# Autodesk Inventor assembly: HalfChassisAssem
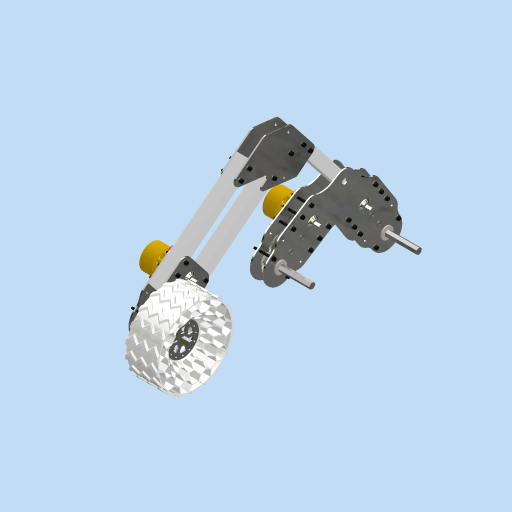
[picture p0: Inventor's stored thumbnail of the model, 512x512]
Saved by Autodesk Inventor 2023 (Build 270158000, 158)
## iProperties
Created: 2023-04-06
Part Number: HalfChassisAssem
Document SubType Name: Assembly
Designer: Dave
Mass: 5362.71 g
Surface Area: 20188.6 cm^2
Volume: 2426.63 cm^3
Density: 2.20995 g/cm^3
Author: Dave
## Documents named in this file (14)
- C:\Github\BehrendURC\CAD\Chassis V3\HalfChassisAssem.iam
- C:\Github\BehrendURC\CAD\Chassis V3\L3 Gearbox Assembly.iam
- C:\Github\BehrendURC\CAD\Chassis V3\L1 Gearbox Assembly.iam
- C:\Github\BehrendURC\CAD\Chassis V3\HipPivotPlate.ipt
- C:\Users\Dave\Documents\GitHub\BehrendURCMechanical\CAD\Chassis V3\aluminumextrusiontool.ipt
- C:\Github\BehrendURC\CAD\Chassis V3\aluminumextrusiontool\aluminumextrusiontool-17-10.6in.ipt
- C:\Github\BehrendURC\CAD\Chassis V3\aluminumextrusiontool\aluminumextrusiontool-17-13.31255in.ipt
- C:\Github\BehrendURC\CAD\Chassis V3\Pivot Files and Assembly\PivotAssembly.iam
- C:\Github\BehrendURC\CAD\Chassis V3\aluminumextrusiontool\aluminumextrusiontool-17-7.9.ipt
- C:\Github\BehrendURC\CAD\Chassis V3\91333A140_Low-Strength Steel Nylon-Insert Locknut.ipt
- C:\Github\BehrendURC\CAD\Chassis V3\90107A011_316 Stainless Steel Washer.ipt
- C:\Github\BehrendURC\CAD\Chassis V3\Bolt Nut Washer assem.iam
- C:\Github\BehrendURC\CAD\Chassis V3\Pivot Files and Assembly\91831A011_18-8 Stainless Steel Nylon-Insert Locknut (1).ipt
- C:\Github\BehrendURC\CAD\Chassis V3\Wheel\WheelAssembly_v9.iam
## Components (20 placed, 12 different names)
1. L3 Gearbox Assembly:1 [sub-assembly] — Mate:4, Tangent:2, Mate:10, Insert:1
2. L1 Gearbox Assembly:1 [sub-assembly] — Flush:2, Flush:3, Mate:1, Flush:6, Mate:2, Flush:7, Mate:3, Mate:11, Flush:13, Tangent:3, Mate:12, Mate:13, Flush:14
3. HipPivotPlate:1 — Flush:3, Flush:4, Flush:5, Mate:5, Insert:4
4. HipPivotPlate:2 — Flush:2, Flush:4, Flush:5, Mate:1, Flush:6, Mate:4, Flush:8, Tangent:1, Mate:6, Flush:9, Insert:6, Insert:7, Insert:9, Insert:10, Insert:11, Insert:12, Insert:14
5. aluminumextrusiontool-17-10.6in:1 — Mate:2, Flush:7, Mate:3
6. aluminumextrusiontool-17-7.9:2 — Mate:5, Flush:8, Tangent:1, Tangent:2, Mate:10
7. aluminumextrusiontool-17-13.31255in:3 — Mate:11, Flush:13, Tangent:3
8. PivotAssembly:2 [sub-assembly] — Insert:1, Insert:16
9. PivotAssembly:3 [sub-assembly] — Insert:6, Insert:15
10. 91333A140_Low-Strength Steel Nylon-Insert Locknut:1 — Insert:5
11. 90107A011_316 Stainless Steel Washer:1 — Insert:4, Insert:5
12. Bolt Nut Washer assem:1 [sub-assembly] — Insert:7
13. Bolt Nut Washer assem:3 [sub-assembly] — Insert:9
14. Bolt Nut Washer assem:4 [sub-assembly] — Insert:10
15. Bolt Nut Washer assem:5 [sub-assembly] — Insert:11
16. Bolt Nut Washer assem:6 [sub-assembly] — Insert:12
17. Bolt Nut Washer assem:8 [sub-assembly] — Insert:14
18. 91831A011_18-8 Stainless Steel Nylon-Insert Locknut (1):1 — Insert:15
19. 91831A011_18-8 Stainless Steel Nylon-Insert Locknut (1):2 — Insert:16
20. WheelAssembly_v9:1 [sub-assembly] — Mate:12, Mate:13, Flush:14
## Relationships (35: Insert 12, Flush 10, Mate 10, Tangent 3)
- Flush:2: L1 Gearbox Assembly:1 ↔ HipPivotPlate:2
- Flush:3: L1 Gearbox Assembly:1 ↔ HipPivotPlate:1
- Flush:4: HipPivotPlate:1 ↔ HipPivotPlate:2
- Flush:5: HipPivotPlate:1 ↔ HipPivotPlate:2
- Mate:1 (396 mm): L1 Gearbox Assembly:1 ↔ HipPivotPlate:2
- Flush:6: L1 Gearbox Assembly:1 ↔ HipPivotPlate:2
- Mate:2: L1 Gearbox Assembly:1 ↔ aluminumextrusiontool-17-10.6in:1
- Flush:7: L1 Gearbox Assembly:1 ↔ aluminumextrusiontool-17-10.6in:1
- Mate:3 (-76.2 mm): L1 Gearbox Assembly:1 ↔ aluminumextrusiontool-17-10.6in:1
- Mate:4 (216 mm): L3 Gearbox Assembly:1 ↔ HipPivotPlate:2
- Mate:5: HipPivotPlate:1 ↔ aluminumextrusiontool-17-7.9:2
- Flush:8: HipPivotPlate:2 ↔ aluminumextrusiontool-17-7.9:2
- Tangent:1 (12.7 mm): HipPivotPlate:2 ↔ aluminumextrusiontool-17-7.9:2
- Tangent:2 (6.35 mm): L3 Gearbox Assembly:1 ↔ aluminumextrusiontool-17-7.9:2
- Mate:6: HipPivotPlate:2
- Flush:9: HipPivotPlate:2
- Mate:10: L3 Gearbox Assembly:1 ↔ aluminumextrusiontool-17-7.9:2
- Mate:11: L1 Gearbox Assembly:1 ↔ aluminumextrusiontool-17-13.31255in:3
- Flush:13: L1 Gearbox Assembly:1 ↔ aluminumextrusiontool-17-13.31255in:3
- Tangent:3 (12.7 mm): L1 Gearbox Assembly:1 ↔ aluminumextrusiontool-17-13.31255in:3
- Insert:1: L3 Gearbox Assembly:1 ↔ PivotAssembly:2
- Insert:4: HipPivotPlate:1 ↔ 90107A011_316 Stainless Steel Washer:1
- Insert:5: 91333A140_Low-Strength Steel Nylon-Insert Locknut:1 ↔ 90107A011_316 Stainless Steel Washer:1
- Insert:6: HipPivotPlate:2 ↔ PivotAssembly:3
- Insert:7: HipPivotPlate:2 ↔ Bolt Nut Washer assem:1
- Insert:9: HipPivotPlate:2 ↔ Bolt Nut Washer assem:3
- Insert:10: HipPivotPlate:2 ↔ Bolt Nut Washer assem:4
- Insert:11: HipPivotPlate:2 ↔ Bolt Nut Washer assem:5
- Insert:12: HipPivotPlate:2 ↔ Bolt Nut Washer assem:6
- Insert:14: HipPivotPlate:2 ↔ Bolt Nut Washer assem:8
- Insert:15: PivotAssembly:3 ↔ 91831A011_18-8 Stainless Steel Nylon-Insert Locknut (1):1
- Insert:16: PivotAssembly:2 ↔ 91831A011_18-8 Stainless Steel Nylon-Insert Locknut (1):2
- Mate:12: L1 Gearbox Assembly:1 ↔ WheelAssembly_v9:1
- Mate:13: L1 Gearbox Assembly:1 ↔ WheelAssembly_v9:1
- Flush:14 (19.05 mm): L1 Gearbox Assembly:1 ↔ WheelAssembly_v9:1
